# Autodesk Inventor assembly: gear_box
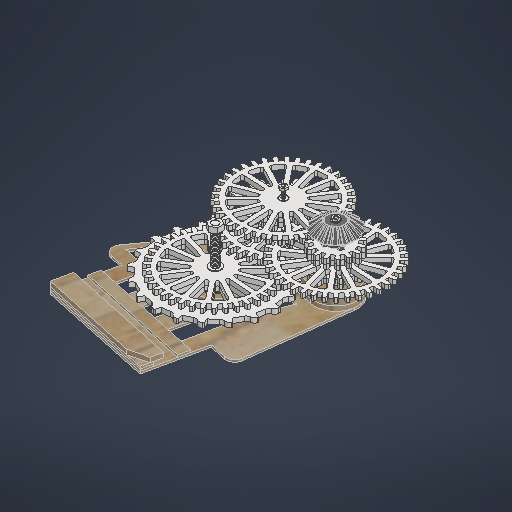
[picture p0: Inventor's stored thumbnail of the model, 512x512]
Saved by Autodesk Inventor 2027.1 (Build 311270010, 270A)
## iProperties
Created: 2025-09-25
Part Number: gear_box
Document SubType Name: Assembly
Designer: hibik
Author: hibik
## Documents named in this file (17)
- D:\model\D2_Conveyor_2026\power_module\gear_box.iam
- D:\model\D2_Conveyor_2026\power_module\gear_box_base.iam
- D:\model\D2_Conveyor_2026\power_module\M3_38.ipt
- D:\model\D2_Conveyor_2026\power_module\roller.ipt
- D:\model\D2_Conveyor_2026\connectors\spacer_22.ipt
- D:\model\D2_Conveyor_2026\power_module\M3_15.ipt
- D:\model\D2_Conveyor_2026\power_module\M3_15_input.ipt
- D:\model\D2_Conveyor_2026\power_module\M3_15_crown_out.ipt
- D:\model\D2_Conveyor_2026\Bearing\bearing_8_12.ipt
- D:\model\D2_Conveyor_2026\power_module\M3_38_holl_small.ipt
- D:\model\D2_Conveyor_2026\power_module\M3_15_hole_small.ipt
- D:\model\D2_Conveyor_2026\Bearing\bearing_4_8.ipt
- D:\model\D2_Conveyor_2026\Bearing\Shaft_Final.ipt
- D:\model\D2_Conveyor_2026\Bearing\Saft_Second.ipt
- D:\model\D2_Conveyor_2026\Bearing\Shaft_First.ipt
- D:\model\D2_Conveyor_2026\Bearing\Spacer_for_Shaft_final_top.ipt
- D:\model\D2_Conveyor_2026\Bearing\Spacer_for_shaft_Second_top.ipt
## Components (31 placed, 16 different names)
1. gear_box_base:1 [sub-assembly] — 挿入:2, フラッシュ:11, フラッシュ:12, フラッシュ:13
2. spacer_22:1 — 挿入:2
3. roller:1 — 回転:1, 回転:2, フラッシュ:1
4. bearing_8_12:1 — 回転:1
5. bearing_8_12:2 — 回転:3
6. M3_15_crown_out:1 — メイト:1, フラッシュ:3, メイト:6, 回転:18
7. M3_15_input:1 — メイト:1, フラッシュ:3, メイト:6, 回転:16, フラッシュ:9
8. M3_38:5 — 回転:4, 回転:5, フラッシュ:7
9. M3_15:5 — 回転:4, 回転:6
10. M3_38:6 — 回転:8, 回転:9, フラッシュ:10
11. M3_15:6 — 回転:7, 回転:8, フラッシュ:2
12. M3_15:7 — 回転:7, フラッシュ:2, 回転:10, フラッシュ:7
13. M3_38:7 — 回転:2, 回転:3, フラッシュ:1
14. bearing_8_12:3 — 回転:5
15. bearing_8_12:4 — 回転:6
16. bearing_8_12:5 — 回転:9
17. bearing_8_12:6 — 回転:10
18. M3_15_hole_small:1 — 回転:13, 回転:14, フラッシュ:8
19. M3_38_holl_small:1 — 回転:12, 回転:13
20. bearing_4_8:1 — 回転:12
21. M3_15_hole_small:2 — リジッド:1, 回転:14, フラッシュ:8, フラッシュ:10
22. bearing_4_8:2 — リジッド:1
23. M3_15_hole_small:3 — 回転:15, 回転:16, フラッシュ:9
24. bearing_4_8:3 — 回転:15
25. Shaft_Final:1 — フラッシュ:11, 回転:17
26. Saft_Second:1 — フラッシュ:12, フラッシュ:14, メイト:8, フラッシュ:15
27. Shaft_First:1 — フラッシュ:13
28. Spacer_for_Shaft_final_top:1 — 回転:17
29. Spacer_for_shaft_Second_top:1 — フラッシュ:14, フラッシュ:15
30. bearing_4_8:5 — 回転:18, 回転:19
31. Spacer_for_shaft_Second_top:2 — 回転:19
## Relationships (35: RevoluteJoint 18, Flush 12, Mate 3, Insert 1, WeldJoint 1)
- 挿入:2 [Insert]: gear_box_base:1 ↔ spacer_22:1
- 回転:1 [RevoluteJoint]: roller:1 ↔ bearing_8_12:1
- メイト:1 [Mate]: M3_15_crown_out:1 ↔ M3_15_input:1
- 回転:2 [RevoluteJoint]: roller:1 ↔ M3_38:7
- 回転:3 [RevoluteJoint]: bearing_8_12:2 ↔ M3_38:7
- フラッシュ:1 [Flush]: roller:1 ↔ M3_38:7
- 回転:4 [RevoluteJoint]: M3_38:5 ↔ M3_15:5
- 回転:5 [RevoluteJoint]: M3_38:5 ↔ bearing_8_12:3
- 回転:6 [RevoluteJoint]: M3_15:5 ↔ bearing_8_12:4
- 回転:7 [RevoluteJoint]: M3_15:6 ↔ M3_15:7
- 回転:8 [RevoluteJoint]: M3_38:6 ↔ M3_15:6
- フラッシュ:2 [Flush]: M3_15:6 ↔ M3_15:7
- 回転:9 [RevoluteJoint]: M3_38:6 ↔ bearing_8_12:5
- 回転:10 [RevoluteJoint]: M3_15:7 ↔ bearing_8_12:6
- フラッシュ:3 [Flush]: M3_15_crown_out:1 ↔ M3_15_input:1
- メイト:6 [Mate]: M3_15_crown_out:1 ↔ M3_15_input:1
- 回転:12 [RevoluteJoint]: M3_38_holl_small:1 ↔ bearing_4_8:1
- 回転:13 [RevoluteJoint]: M3_15_hole_small:1 ↔ M3_38_holl_small:1
- フラッシュ:7 [Flush]: M3_38:5 ↔ M3_15:7
- リジッド:1 [WeldJoint]: M3_15_hole_small:2 ↔ bearing_4_8:2
- 回転:14 [RevoluteJoint]: M3_15_hole_small:1 ↔ M3_15_hole_small:2
- フラッシュ:8 [Flush]: M3_15_hole_small:1 ↔ M3_15_hole_small:2
- 回転:15 [RevoluteJoint]: M3_15_hole_small:3 ↔ bearing_4_8:3
- 回転:16 [RevoluteJoint]: M3_15_input:1 ↔ M3_15_hole_small:3
- フラッシュ:9 [Flush]: M3_15_input:1 ↔ M3_15_hole_small:3
- フラッシュ:10 [Flush]: M3_38:6 ↔ M3_15_hole_small:2
- フラッシュ:11 [Flush]: gear_box_base:1 ↔ Shaft_Final:1
- フラッシュ:12 [Flush]: gear_box_base:1 ↔ Saft_Second:1
- フラッシュ:13 [Flush]: gear_box_base:1 ↔ Shaft_First:1
- 回転:17 [RevoluteJoint]: Shaft_Final:1 ↔ Spacer_for_Shaft_final_top:1
- フラッシュ:14 [Flush]: Saft_Second:1 ↔ Spacer_for_shaft_Second_top:1
- メイト:8 [Mate]: Saft_Second:1
- フラッシュ:15 [Flush]: Saft_Second:1 ↔ Spacer_for_shaft_Second_top:1
- 回転:18 [RevoluteJoint]: M3_15_crown_out:1 ↔ bearing_4_8:5
- 回転:19 [RevoluteJoint]: bearing_4_8:5 ↔ Spacer_for_shaft_Second_top:2
